# Autodesk Inventor assembly: test_stand
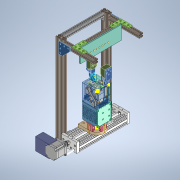
[picture p0: Inventor's stored thumbnail of the model, 180x180]
Saved by Autodesk Inventor 2022 (Build 260153000, 153)
## iProperties
Created: 2022-01-11
Part Number: test_stand
Document SubType Name: Assembly
Designer: kylem
Author: kylem
## Documents named in this file (12)
- C:\Users\kylem\OneDrive\Documents\GitHub\Gripper_Hardware\test_stand\test_stand.iam
- C:\Users\kylem\Downloads\C-Beam Linear Actuator 250mm.ipt
- C:\Users\kylem\OneDrive\Documents\GitHub\Gripper_Hardware\Gripper_Design_NonCompliant_No_UR5.iam
- C:\Users\kylem\Downloads\5537T408_T-Slotted Framing.ipt
- C:\Users\kylem\Downloads\5537T104_T-Slotted Framing.ipt
- C:\Users\kylem\Downloads\5537T962_T-Slotted Framing.ipt
- C:\Users\kylem\Downloads\3136N922_T-Slotted Framing.ipt
- C:\Users\kylem\OneDrive\Documents\GitHub\Gripper_Hardware\test_stand\rivet_material.ipt
- C:\Users\kylem\Downloads\97482A070_Aluminum Domed Head Solid Rivets.ipt
- C:\Users\kylem\OneDrive\Documents\GitHub\Gripper_Hardware\test_stand\motor_support.ipt
- C:\Users\kylem\Downloads\5537T935_T-Slotted Framing.ipt
- C:\Users\kylem\Downloads\5537T939_T-Slotted Framing.ipt
## Components (29 placed, 11 different names)
1. C-Beam Linear Actuator 250mm:1 — Flush:4, Flush:6, Mate:54, Mate:55, Mate:56, Mate:58, Flush:26, Mate:69, Mate:71, Flush:27, Flush:28, Mate:72, Mate:73
2. Gripper_Design_NonCompliant_No_UR5:1 [sub-assembly] — Mate:58, Flush:26
3. 5537T408_T-Slotted Framing:1 — Flush:4, Mate:12, Mate:13, Mate:60, Flush:25, Mate:70, Flush:27, Mate:73, Flush:31, Flush:32
4. 5537T408_T-Slotted Framing:2 — Flush:6, Mate:9, Mate:10, Mate:59, Mate:62, Mate:68, Flush:28, Mate:72, Flush:29
5. 5537T104_T-Slotted Framing:1 — Mate:26, Mate:27, Flush:21, Flush:22, Mate:28, Mate:29, Flush:23, Mate:64, Mate:66
6. 5537T962_T-Slotted Framing:1 — Mate:9, Mate:10, Flush:8, Mate:22, Flush:17
7. 5537T104_T-Slotted Framing:2 — Flush:8, Mate:22, Flush:17, Mate:23, Flush:18, Mate:26
8. 5537T962_T-Slotted Framing:2 — Mate:12, Mate:13, Flush:15, Mate:24, Flush:19
9. 5537T104_T-Slotted Framing:3 — Flush:15, Mate:24, Flush:19, Mate:25, Flush:20, Mate:43
10. 3136N922_T-Slotted Framing:1 — Mate:23, Flush:18, Mate:27, Flush:21
11. 3136N922_T-Slotted Framing:2 — Mate:25, Flush:20, Flush:22, Mate:28
12. rivet_material:1 — Mate:29, Flush:23, Mate:32, Mate:33, Mate:34, Mate:35, Mate:36, Mate:37, Mate:38, Mate:39, Mate:40, Mate:41, Mate:42, Mate:43, Mate:44, Mate:45, Mate:46, Mate:47, Mate:48, Mate:49, Mate:50, Mate:51, Mate:52, Mate:53, Angle:1, Mate:65, Mate:67
13. 97482A070_Aluminum Domed Head Solid Rivets:1 — Mate:32, Mate:41, Mate:44
14. 97482A070_Aluminum Domed Head Solid Rivets:8 — Mate:36, Mate:52
15. 97482A070_Aluminum Domed Head Solid Rivets:9 — Mate:33, Mate:51
16. 97482A070_Aluminum Domed Head Solid Rivets:10 — Mate:34, Mate:48
17. 97482A070_Aluminum Domed Head Solid Rivets:11 — Mate:35, Mate:46
18. 97482A070_Aluminum Domed Head Solid Rivets:12 — Mate:37, Mate:42, Mate:45
19. 97482A070_Aluminum Domed Head Solid Rivets:13 — Mate:38, Mate:50, Mate:53
20. 97482A070_Aluminum Domed Head Solid Rivets:14 — Mate:39, Mate:49
21. 97482A070_Aluminum Domed Head Solid Rivets:15 — Mate:40, Mate:47
22. motor_support:1 — Mate:54, Mate:55, Mate:56
23. 5537T104_T-Slotted Framing:4 — Mate:59, Mate:61, Flush:25, Mate:63, Flush:29, Flush:30, Flush:32
24. 5537T935_T-Slotted Framing:1 — Mate:60, Mate:61, Flush:31
25. 5537T935_T-Slotted Framing:2 — Mate:62, Mate:63, Flush:30
26. 5537T935_T-Slotted Framing:3 — Mate:64, Angle:1, Mate:65
27. 5537T935_T-Slotted Framing:4 — Mate:66, Mate:67
28. 5537T939_T-Slotted Framing:1 — Mate:68, Mate:69
29. 5537T939_T-Slotted Framing:2 — Mate:70, Mate:71
## Relationships (73: Mate 53, Flush 19, Angle 1)
- Flush:4: C-Beam Linear Actuator 250mm:1 ↔ 5537T408_T-Slotted Framing:1
- Flush:6: C-Beam Linear Actuator 250mm:1 ↔ 5537T408_T-Slotted Framing:2
- Mate:9: 5537T408_T-Slotted Framing:2 ↔ 5537T962_T-Slotted Framing:1
- Mate:10 (-20 mm): 5537T408_T-Slotted Framing:2 ↔ 5537T962_T-Slotted Framing:1
- Flush:8 (20 mm): 5537T962_T-Slotted Framing:1 ↔ 5537T104_T-Slotted Framing:2
- Mate:12: 5537T408_T-Slotted Framing:1 ↔ 5537T962_T-Slotted Framing:2
- Mate:13 (-20 mm): 5537T408_T-Slotted Framing:1 ↔ 5537T962_T-Slotted Framing:2
- Flush:15 (20 mm): 5537T962_T-Slotted Framing:2 ↔ 5537T104_T-Slotted Framing:3
- Mate:22: 5537T962_T-Slotted Framing:1 ↔ 5537T104_T-Slotted Framing:2
- Flush:17: 5537T962_T-Slotted Framing:1 ↔ 5537T104_T-Slotted Framing:2
- Mate:23: 5537T104_T-Slotted Framing:2 ↔ 3136N922_T-Slotted Framing:1
- Flush:18 (0.5 mm): 5537T104_T-Slotted Framing:2 ↔ 3136N922_T-Slotted Framing:1
- Mate:24: 5537T962_T-Slotted Framing:2 ↔ 5537T104_T-Slotted Framing:3
- Flush:19: 5537T962_T-Slotted Framing:2 ↔ 5537T104_T-Slotted Framing:3
- Mate:25: 5537T104_T-Slotted Framing:3 ↔ 3136N922_T-Slotted Framing:2
- Flush:20 (0.5 mm): 5537T104_T-Slotted Framing:3 ↔ 3136N922_T-Slotted Framing:2
- Mate:26: 5537T104_T-Slotted Framing:1 ↔ 5537T104_T-Slotted Framing:2
- Mate:27: 5537T104_T-Slotted Framing:1 ↔ 3136N922_T-Slotted Framing:1
- Flush:21 (0.5 mm): 5537T104_T-Slotted Framing:1 ↔ 3136N922_T-Slotted Framing:1
- Flush:22 (0.5 mm): 5537T104_T-Slotted Framing:1 ↔ 3136N922_T-Slotted Framing:2
- Mate:28: 5537T104_T-Slotted Framing:1 ↔ 3136N922_T-Slotted Framing:2
- Mate:29: 5537T104_T-Slotted Framing:1 ↔ rivet_material:1
- Flush:23: 5537T104_T-Slotted Framing:1 ↔ rivet_material:1
- Mate:32: rivet_material:1 ↔ 97482A070_Aluminum Domed Head Solid Rivets:1
- Mate:33: rivet_material:1 ↔ 97482A070_Aluminum Domed Head Solid Rivets:9
- Mate:34: rivet_material:1 ↔ 97482A070_Aluminum Domed Head Solid Rivets:10
- Mate:35: rivet_material:1 ↔ 97482A070_Aluminum Domed Head Solid Rivets:11
- Mate:36: rivet_material:1 ↔ 97482A070_Aluminum Domed Head Solid Rivets:8
- Mate:37: rivet_material:1 ↔ 97482A070_Aluminum Domed Head Solid Rivets:12
- Mate:38: rivet_material:1 ↔ 97482A070_Aluminum Domed Head Solid Rivets:13
- Mate:39: rivet_material:1 ↔ 97482A070_Aluminum Domed Head Solid Rivets:14
- Mate:40: rivet_material:1 ↔ 97482A070_Aluminum Domed Head Solid Rivets:15
- Mate:41 (-30 mm): rivet_material:1 ↔ 97482A070_Aluminum Domed Head Solid Rivets:1
- Mate:42 (-43 mm): rivet_material:1 ↔ 97482A070_Aluminum Domed Head Solid Rivets:12
- Mate:43: 5537T104_T-Slotted Framing:3 ↔ rivet_material:1
- Mate:44 (-25 mm): rivet_material:1 ↔ 97482A070_Aluminum Domed Head Solid Rivets:1
- Mate:45 (-25 mm): rivet_material:1 ↔ 97482A070_Aluminum Domed Head Solid Rivets:12
- Mate:46 (-25 mm): rivet_material:1 ↔ 97482A070_Aluminum Domed Head Solid Rivets:11
- Mate:47 (-25 mm): rivet_material:1 ↔ 97482A070_Aluminum Domed Head Solid Rivets:15
- Mate:48 (-25 mm): rivet_material:1 ↔ 97482A070_Aluminum Domed Head Solid Rivets:10
- Mate:49 (-25 mm): rivet_material:1 ↔ 97482A070_Aluminum Domed Head Solid Rivets:14
- Mate:50 (-25 mm): rivet_material:1 ↔ 97482A070_Aluminum Domed Head Solid Rivets:13
- Mate:51 (-25 mm): rivet_material:1 ↔ 97482A070_Aluminum Domed Head Solid Rivets:9
- Mate:52 (-25 mm): rivet_material:1 ↔ 97482A070_Aluminum Domed Head Solid Rivets:8
- Mate:53 (-56 mm): rivet_material:1 ↔ 97482A070_Aluminum Domed Head Solid Rivets:13
- Mate:54: C-Beam Linear Actuator 250mm:1 ↔ motor_support:1
- Mate:55 (2 mm): C-Beam Linear Actuator 250mm:1 ↔ motor_support:1
- Mate:56: C-Beam Linear Actuator 250mm:1 ↔ motor_support:1
- Mate:58: C-Beam Linear Actuator 250mm:1 ↔ Gripper_Design_NonCompliant_No_UR5:1
- Mate:59: 5537T408_T-Slotted Framing:2 ↔ 5537T104_T-Slotted Framing:4
- Mate:60: 5537T408_T-Slotted Framing:1 ↔ 5537T935_T-Slotted Framing:1
- Mate:61: 5537T104_T-Slotted Framing:4 ↔ 5537T935_T-Slotted Framing:1
- Flush:25: 5537T408_T-Slotted Framing:1 ↔ 5537T104_T-Slotted Framing:4
- Mate:62: 5537T408_T-Slotted Framing:2 ↔ 5537T935_T-Slotted Framing:2
- Mate:63: 5537T104_T-Slotted Framing:4 ↔ 5537T935_T-Slotted Framing:2
- Mate:64: 5537T104_T-Slotted Framing:1 ↔ 5537T935_T-Slotted Framing:3
- Angle:1 (180 deg): rivet_material:1 ↔ 5537T935_T-Slotted Framing:3
- Mate:65: rivet_material:1 ↔ 5537T935_T-Slotted Framing:3
- Mate:66: 5537T104_T-Slotted Framing:1 ↔ 5537T935_T-Slotted Framing:4
- Mate:67: rivet_material:1 ↔ 5537T935_T-Slotted Framing:4
- Flush:26 (-30.38 mm): C-Beam Linear Actuator 250mm:1 ↔ Gripper_Design_NonCompliant_No_UR5:1
- Mate:68: 5537T408_T-Slotted Framing:2 ↔ 5537T939_T-Slotted Framing:1
- Mate:69: C-Beam Linear Actuator 250mm:1 ↔ 5537T939_T-Slotted Framing:1
- Mate:70: 5537T408_T-Slotted Framing:1 ↔ 5537T939_T-Slotted Framing:2
- Mate:71: C-Beam Linear Actuator 250mm:1 ↔ 5537T939_T-Slotted Framing:2
- Flush:27 (-9.5 mm): C-Beam Linear Actuator 250mm:1 ↔ 5537T408_T-Slotted Framing:1
- Flush:28 (-9.5 mm): C-Beam Linear Actuator 250mm:1 ↔ 5537T408_T-Slotted Framing:2
- Mate:72: C-Beam Linear Actuator 250mm:1 ↔ 5537T408_T-Slotted Framing:2
- Mate:73: C-Beam Linear Actuator 250mm:1 ↔ 5537T408_T-Slotted Framing:1
- Flush:29: 5537T408_T-Slotted Framing:2 ↔ 5537T104_T-Slotted Framing:4
- Flush:30: 5537T104_T-Slotted Framing:4 ↔ 5537T935_T-Slotted Framing:2
- Flush:31: 5537T408_T-Slotted Framing:1 ↔ 5537T935_T-Slotted Framing:1
- Flush:32: 5537T408_T-Slotted Framing:1 ↔ 5537T104_T-Slotted Framing:4
